# Autodesk Inventor assembly: TZ V6 Hotend
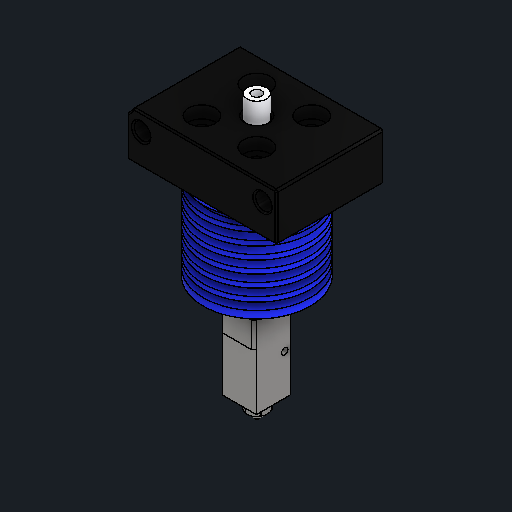
[picture p0: Inventor's stored thumbnail of the model, 512x512]
Saved by Autodesk Inventor 2026.1 (Build 301233020, 233B)
## iProperties
Created: 2025-11-13
Part Number: TZ V6 Hotend
Document SubType Name: Assembly
Designer: JoshuaEah
Author: JoshuaEah
## Documents named in this file (8)
- C:\Users\JoshuaEah\Documents\GitHub\Voron-0\CAD\Toolhead\Subassemblies\TZ V6 Hotend.iam
- C:\Users\JoshuaEah\Documents\GitHub\Voron-0\CAD\Toolhead\Parts\Hotend\Radiator.ipt
- C:\Users\JoshuaEah\Documents\GitHub\Voron-0\CAD\Toolhead\Parts\Hotend\Heatbrake.ipt
- C:\Users\JoshuaEah\Documents\GitHub\Voron-0\CAD\Toolhead\Parts\Hotend\Heatblock.ipt
- C:\Users\JoshuaEah\Documents\GitHub\Voron-0\CAD\Toolhead\Parts\Hotend\Nozzle.ipt
- C:\Users\JoshuaEah\Documents\GitHub\Voron-0\CAD\Hardware\Fasteners\M1.6x6 SHCS.ipt
- C:\Users\JoshuaEah\Documents\GitHub\Voron-0\CAD\Toolhead\Parts\Hotend\Formbot Mount.ipt
- C:\Users\JoshuaEah\Documents\GitHub\Voron-0\CAD\Toolhead\Parts\Hotend\PTFE Tube.ipt
## Components (8 placed, 7 different names)
1. Radiator:1 — Insert:1, Insert:2, Insert:7, Insert:8
2. Heatbrake:1 — Insert:4
3. Heatblock:1 — Insert:1, Insert:2, Insert:3, Insert:4, Insert:5, Insert:6
4. Nozzle:1 — Insert:3
5. M1.6x6 SHCS:1 — Insert:5
6. M1.6x6 SHCS:2 — Insert:6
7. Formbot Mount:1 — Insert:7, Insert:8, Mate:1, Flush:1
8. PTFE Tube:1 — Mate:1, Flush:1
## Relationships (10: Insert 8, Mate 1, Flush 1)
- Insert:1: Radiator:1 ↔ Heatblock:1
- Insert:2: Radiator:1 ↔ Heatblock:1
- Insert:3: Heatblock:1 ↔ Nozzle:1
- Insert:4: Heatbrake:1 ↔ Heatblock:1
- Insert:5: Heatblock:1 ↔ M1.6x6 SHCS:1
- Insert:6: Heatblock:1 ↔ M1.6x6 SHCS:2
- Insert:7: Radiator:1 ↔ Formbot Mount:1
- Insert:8: Radiator:1 ↔ Formbot Mount:1
- Mate:1: Formbot Mount:1 ↔ PTFE Tube:1
- Flush:1 (-4 mm): Formbot Mount:1 ↔ PTFE Tube:1
